# Autodesk Inventor assembly: Storage System Assembly
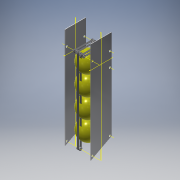
[picture p0: Inventor's stored thumbnail of the model, 180x180]
Saved by Autodesk Inventor 2019.4 (Build 234330000, 330)
## iProperties
Created: 2020-01-24
Part Number: Storage System Assembly
Document SubType Name: Assembly
Designer: admin
Author: admin
## Documents named in this file (8)
- C:\Users\admin\Desktop\FRC 2020 Engineering\GitHub\7738-2020\Robot V2\Storage System\Storage System Assembly.iam
- C:\Users\admin\Desktop\FRC 2020 Engineering\GitHub\7738-2020\Robot V2\Storage System\Storage Side Plate.ipt
- C:\Users\admin\Desktop\FRC 2020 Engineering\GitHub\7738-2020\Robot V2\Storage System\Storage System Assembly\Design Accelerator\Synchronous Belts Transmission1.iam
- C:\Users\admin\Desktop\FRC 2020 Engineering\GitHub\7738-2020\Robot V2\Storage System\Storage System Assembly\Design Accelerator\Synchronous Belts Transmission3.iam
- C:\Users\admin\Desktop\FRC 2020 Engineering\GitHub\7738-2020\Robot V2\Storage System\Storage System Assembly\Design Accelerator\Synchronous Belts Transmission4.iam
- C:\Users\admin\Desktop\FRC 2020 Engineering\GitHub\7738-2020\Robot V2\Storage System\Storage System Assembly\Design Accelerator\Synchronous Belts Transmission5.iam
- C:\Users\admin\Desktop\FRC 2020 Engineering\GitHub\7738-2020\Robot V2\Storage System\Storage System Assembly\Design Accelerator\Synchronous Belts Transmission6.iam
- C:\Users\admin\Desktop\FRC 2020 Engineering\GitHub\7738-2020\Power Cell.ipt
## Components (11 placed, 3 different names)
1. Storage Side Plate:1 — Mate:1, Mate:2, Mate:3, Flush:2
2. Storage Side Plate:2 — Mate:1, Mate:2, Flush:1, Mate:12
3. Synchronous Belts Transmission:1 [sub-assembly]
4. Synchronous Belts Transmission:2 [sub-assembly]
5. Synchronous Belts Transmission:3 [sub-assembly]
6. Synchronous Belts Transmission:4 [sub-assembly]
7. Synchronous Belts Transmission:5 [sub-assembly]
8. Power Cell:1 — Mate:4, Mate:8
9. Power Cell:2 — Mate:5, Mate:11
10. Power Cell:3 — Mate:6, Mate:9
11. Power Cell:4 — Mate:7, Mate:10
## Relationships (14: Mate 12, Flush 2)
- Mate:1: Storage Side Plate:1 ↔ Storage Side Plate:2
- Mate:2: Storage Side Plate:1 ↔ Storage Side Plate:2
- Mate:3 (114.3 mm): Storage Side Plate:1
- Flush:1 (114.3 mm): Storage Side Plate:2
- Mate:4: Power Cell:1
- Mate:5: Power Cell:2
- Mate:6: Power Cell:3
- Mate:7: Power Cell:4
- Mate:8: Power Cell:1
- Mate:9: Power Cell:3
- Mate:10: Power Cell:4
- Mate:11: Power Cell:2
- Mate:12: Storage Side Plate:2
- Flush:2: Storage Side Plate:1
